# Autodesk Inventor assembly: V4Slapper
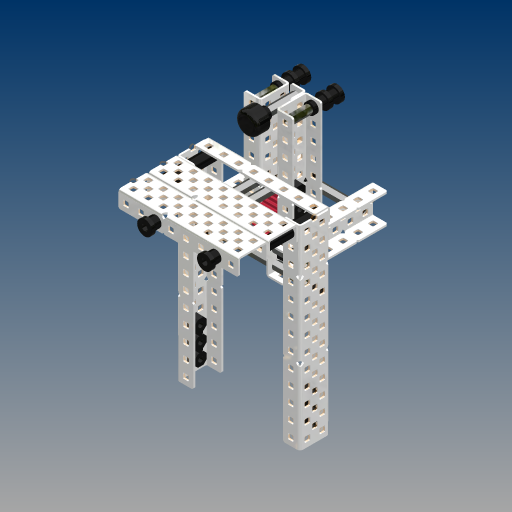
[picture p0: Inventor's stored thumbnail of the model, 512x512]
Saved by Autodesk Inventor 2023 (Build 270158000, 158)
## iProperties
Created: 2024-01-13
Part Number: V4Slapper
Document SubType Name: Assembly
Designer: eddie
Author: eddie
## Documents named in this file (24)
- C:\Users\eddie\Documents\81208X-Over-Under-CAD\V4\V4Slapper.iam
- C:\Users\eddie\Documents\81208X-Over-Under-CAD\VEX-CAD-Inventor-1.4.0\Structure\C Channel\Aluminum 1x2x1\Alu C 1x2x1x13.ipt
- C:\Users\eddie\Documents\81208X-Over-Under-CAD\VEX-CAD-Inventor-1.4.0\Motion\Spacers\Spacer Nylon .375 OD\NSpacer .375 OD x .500.ipt
- C:\Users\eddie\Documents\81208X-Over-Under-CAD\VEX-CAD-Inventor-1.4.0\Motion\Spacers\Spacer Nylon .375 OD.ipt
- C:\Users\eddie\Documents\81208X-Over-Under-CAD\VEX-CAD-Inventor-1.4.0\Structure\Standoff\Standoff 3.00.ipt
- C:\Users\eddie\Documents\81208X-Over-Under-CAD\VEX-CAD-Inventor-1.4.0\Structure\Standoff.ipt
- C:\Users\eddie\Documents\81208X-Over-Under-CAD\VEX-CAD-Inventor-1.4.0\Motion\Spacers\Spacer Nylon .375 OD\NSpacer .375 OD x .375.ipt
- C:\Users\eddie\Documents\81208X-Over-Under-CAD\VEX-CAD-Inventor-1.4.0\Structure\Angle\Aluminum\1x1\Alu Angle 1x1x8.ipt
- C:\Users\eddie\Documents\81208X-Over-Under-CAD\VEX-CAD-Inventor-1.4.0\Structure\C Channel\Aluminum 1x2x1\Alu C 1x2x1x8.ipt
- C:\Users\eddie\Documents\81208X-Over-Under-CAD\VEX-CAD-Inventor-1.4.0\Motion\Spacers\Spacer Nylon .375 OD\NSpacer .375 OD x .250.ipt
- C:\Users\eddie\Documents\81208X-Over-Under-CAD\VEX-CAD-Inventor-1.4.0\Motion\Spacers\Spacer Nylon .500 OD\NSpacer Black .500 OD x .125.ipt
- C:\Users\eddie\Documents\81208X-Over-Under-CAD\VEX-CAD-Inventor-1.4.0\Motion\Spacers\Spacer Nylon .500 OD.ipt
- C:\Users\eddie\Documents\81208X-Over-Under-CAD\VEX-CAD-Inventor-1.4.0\Motion\Shaft LS\Bearing Flat.ipt
- C:\Users\eddie\Documents\81208X-Over-Under-CAD\VEX-CAD-Inventor-1.4.0\Structure\Standoff\Standoff 1.00.ipt
- C:\Users\eddie\Documents\81208X-Over-Under-CAD\VEX-CAD-Inventor-1.4.0\Structure\C Channel\Aluminum 1x2x1\Alu C 1x2x1x7.ipt
- C:\Users\eddie\Documents\81208X-Over-Under-CAD\VEX-CAD-Inventor-1.4.0\Motion\Spacers\Washer Steel\SWasher .375 OD x .031250.ipt
- C:\Users\eddie\Documents\81208X-Over-Under-CAD\VEX-CAD-Inventor-1.4.0\Motion\Spacers\Washer Steel.ipt
- C:\Users\eddie\Documents\81208X-Over-Under-CAD\VEX-CAD-Inventor-1.4.0\Motion\Spacers\Spacer Nylon .375 OD\NSpacer .375 OD x .125.ipt
- C:\Users\eddie\Documents\81208X-Over-Under-CAD\VEX-CAD-Inventor-1.4.0\Structure\Standoff\Standoff 1.50.ipt
- C:\Users\eddie\Documents\81208X-Over-Under-CAD\VEX-CAD-Inventor-1.4.0\Motion\Gears\HS Gear\HS 36T Gear, Square.iam
- C:\Users\eddie\Documents\81208X-Over-Under-CAD\VEX-CAD-Inventor-1.4.0\Motion\Gears\HS Gear.iam
- C:\Users\eddie\Documents\81208X-Over-Under-CAD\VEX-CAD-Inventor-1.4.0\Structure\Standoff\Standoff .75.ipt
- C:\Users\eddie\Documents\81208X-Over-Under-CAD\VEX-CAD-Inventor-1.4.0\Structure\Angle\Aluminum\1x1\Alu Angle 1x1x3.ipt
- C:\Users\eddie\Documents\81208X-Over-Under-CAD\VEX-CAD-Inventor-1.4.0\Structure\Hardware\Rubber Bumper Threaded.ipt
## Components (61 placed, 18 different names)
1. Alu C 1x2x1x13:1 — Insert:2, Insert:5, Insert:9, Insert:10, Insert:22, Insert:25, Insert:26
2. Alu C 1x2x1x13:2 — Insert:1, Insert:6, Insert:20, Insert:21, Insert:23, Insert:24
3. NSpacer .375 OD x .500:1 — Insert:1, Insert:3
4. NSpacer .375 OD x .500:2 — Insert:2, Insert:4
5. Standoff 3.00:1 — Insert:3, Insert:4
6. NSpacer .375 OD x .500:3 — Insert:6, Insert:7
7. NSpacer .375 OD x .500:4 — Insert:5, Insert:8
8. NSpacer .375 OD x .375:5 — Insert:7
9. NSpacer .375 OD x .375:6 — Insert:8
10. Alu Angle 1x1x8:1 — Insert:9, Insert:27, Insert:28
11. Alu C 1x2x1x8:1 — Insert:10, Insert:11, Insert:12, Insert:14
12. Alu C 1x2x1x8:2 — Insert:11, Insert:16, Insert:17
13. NSpacer .375 OD x .500:7 — Insert:12, Insert:13
14. NSpacer .375 OD x .375:8 — Insert:13
15. NSpacer .375 OD x .500:9 — Insert:14, Insert:15
16. NSpacer .375 OD x .375:10 — Insert:15
17. NSpacer .375 OD x .250:11 — Insert:17, Insert:19
18. NSpacer .375 OD x .250:12 — Insert:16, Insert:18
19. NSpacer Black .500 OD x .125:1 — Insert:19
20. NSpacer Black .500 OD x .125:2 — Insert:18
21. Bearing Flat:1 — Insert:20, Insert:21
22. Bearing Flat:2 — Insert:22
23. Standoff 1.00:2 — Insert:24
24. Standoff 1.00:3 — Insert:23, Insert:30
25. Standoff 1.00:4 — Insert:25, Insert:29
26. Standoff 1.00:5 — Insert:26
27. Standoff 1.00:6 — Insert:28
28. Standoff 1.00:7 — Insert:27
29. Alu C 1x2x1x7:1 — Insert:30, Insert:33, Insert:35, Insert:44
30. Alu C 1x2x1x7:2 — Insert:29, Insert:32, Insert:34, Insert:43
31. Bearing Flat:4 — Insert:32
32. Bearing Flat:5 — Insert:33
33. SWasher .375 OD x .031250:1 — Insert:34, Insert:36
34. SWasher .375 OD x .031250:2 — Insert:35, Insert:37
35. NSpacer .375 OD x .125:13 — Insert:37, Insert:38
36. NSpacer .375 OD x .125:14 — Insert:36
37. Standoff 1.50:8 — Insert:38, Insert:39
38. NSpacer .375 OD x .125:15 — Insert:39
39. Alu C 1x2x1x8:3 — Insert:46, Insert:48, Insert:50, Insert:60, Insert:67
40. Alu C 1x2x1x8:4 — Insert:42, Insert:49, Insert:59
41. Bearing Flat:6 — Insert:42, Insert:45
42. NSpacer .375 OD x .375:18 — Insert:43, Insert:47
43. NSpacer .375 OD x .375:19 — Insert:44, Insert:45
44. Bearing Flat:7 — Insert:46, Insert:47
45. HS 36T Gear, Square:1 [sub-assembly] — Insert:48
46. Standoff .75:9 — Insert:50, Insert:52
47. Standoff .75:10 — Insert:49, Insert:51
48. NSpacer .375 OD x .125:20 — Insert:51
49. NSpacer .375 OD x .125:21 — Insert:52
50. NSpacer Black .500 OD x .125:5 — Insert:61, Insert:63
51. NSpacer Black .500 OD x .125:6 — Insert:62, Insert:64
52. NSpacer .375 OD x .250:26 — Insert:59, Insert:62
53. NSpacer .375 OD x .250:27 — Insert:60, Insert:61
54. NSpacer .375 OD x .250:28 — Insert:63, Insert:65
55. NSpacer .375 OD x .250:29 — Insert:64, Insert:66
56. NSpacer Black .500 OD x .125:7 — Insert:65
57. NSpacer Black .500 OD x .125:8 — Insert:66
58. Alu Angle 1x1x3:1 — Insert:67, Insert:68
59. Standoff 1.00:11 — Insert:68, Insert:69
60. NSpacer .375 OD x .250:30 — Insert:69, Insert:70
61. Rubber Bumper Threaded:1 — Insert:70
## Relationships (61: Insert 61)
- Insert:1: Alu C 1x2x1x13:2 ↔ NSpacer .375 OD x .500:1
- Insert:2: Alu C 1x2x1x13:1 ↔ NSpacer .375 OD x .500:2
- Insert:3: NSpacer .375 OD x .500:1 ↔ Standoff 3.00:1
- Insert:4: NSpacer .375 OD x .500:2 ↔ Standoff 3.00:1
- Insert:5: Alu C 1x2x1x13:1 ↔ NSpacer .375 OD x .500:4
- Insert:6: Alu C 1x2x1x13:2 ↔ NSpacer .375 OD x .500:3
- Insert:7: NSpacer .375 OD x .500:3 ↔ NSpacer .375 OD x .375:5
- Insert:8: NSpacer .375 OD x .500:4 ↔ NSpacer .375 OD x .375:6
- Insert:9: Alu C 1x2x1x13:1 ↔ Alu Angle 1x1x8:1
- Insert:10: Alu C 1x2x1x13:1 ↔ Alu C 1x2x1x8:1
- Insert:11: Alu C 1x2x1x8:1 ↔ Alu C 1x2x1x8:2
- Insert:12: Alu C 1x2x1x8:1 ↔ NSpacer .375 OD x .500:7
- Insert:13: NSpacer .375 OD x .500:7 ↔ NSpacer .375 OD x .375:8
- Insert:14: Alu C 1x2x1x8:1 ↔ NSpacer .375 OD x .500:9
- Insert:15: NSpacer .375 OD x .500:9 ↔ NSpacer .375 OD x .375:10
- Insert:16: Alu C 1x2x1x8:2 ↔ NSpacer .375 OD x .250:12
- Insert:17: Alu C 1x2x1x8:2 ↔ NSpacer .375 OD x .250:11
- Insert:18: NSpacer .375 OD x .250:12 ↔ NSpacer Black .500 OD x .125:2
- Insert:19: NSpacer .375 OD x .250:11 ↔ NSpacer Black .500 OD x .125:1
- Insert:20: Alu C 1x2x1x13:2 ↔ Bearing Flat:1
- Insert:21: Alu C 1x2x1x13:2 ↔ Bearing Flat:1
- Insert:22: Alu C 1x2x1x13:1 ↔ Bearing Flat:2
- Insert:23: Alu C 1x2x1x13:2 ↔ Standoff 1.00:3
- Insert:24: Alu C 1x2x1x13:2 ↔ Standoff 1.00:2
- Insert:25: Alu C 1x2x1x13:1 ↔ Standoff 1.00:4
- Insert:26: Alu C 1x2x1x13:1 ↔ Standoff 1.00:5
- Insert:27: Alu Angle 1x1x8:1 ↔ Standoff 1.00:7
- Insert:28: Alu Angle 1x1x8:1 ↔ Standoff 1.00:6
- Insert:29: Standoff 1.00:4 ↔ Alu C 1x2x1x7:2
- Insert:30: Standoff 1.00:3 ↔ Alu C 1x2x1x7:1
- Insert:32: Alu C 1x2x1x7:2 ↔ Bearing Flat:4
- Insert:33: Alu C 1x2x1x7:1 ↔ Bearing Flat:5
- Insert:34: Alu C 1x2x1x7:2 ↔ SWasher .375 OD x .031250:1
- Insert:35: Alu C 1x2x1x7:1 ↔ SWasher .375 OD x .031250:2
- Insert:36: SWasher .375 OD x .031250:1 ↔ NSpacer .375 OD x .125:14
- Insert:37: SWasher .375 OD x .031250:2 ↔ NSpacer .375 OD x .125:13
- Insert:38: NSpacer .375 OD x .125:13 ↔ Standoff 1.50:8
- Insert:39: Standoff 1.50:8 ↔ NSpacer .375 OD x .125:15
- Insert:42: Alu C 1x2x1x8:4 ↔ Bearing Flat:6
- Insert:43: Alu C 1x2x1x7:2 ↔ NSpacer .375 OD x .375:18
- Insert:44: Alu C 1x2x1x7:1 ↔ NSpacer .375 OD x .375:19
- Insert:45: Bearing Flat:6 ↔ NSpacer .375 OD x .375:19
- Insert:46: Alu C 1x2x1x8:3 ↔ Bearing Flat:7
- Insert:47: NSpacer .375 OD x .375:18 ↔ Bearing Flat:7
- Insert:48: Alu C 1x2x1x8:3 ↔ HS 36T Gear, Square:1
- Insert:49: Alu C 1x2x1x8:4 ↔ Standoff .75:10
- Insert:50: Alu C 1x2x1x8:3 ↔ Standoff .75:9
- Insert:51: Standoff .75:10 ↔ NSpacer .375 OD x .125:20
- Insert:52: Standoff .75:9 ↔ NSpacer .375 OD x .125:21
- Insert:59: Alu C 1x2x1x8:4 ↔ NSpacer .375 OD x .250:26
- Insert:60: Alu C 1x2x1x8:3 ↔ NSpacer .375 OD x .250:27
- Insert:61: NSpacer Black .500 OD x .125:5 ↔ NSpacer .375 OD x .250:27
- Insert:62: NSpacer Black .500 OD x .125:6 ↔ NSpacer .375 OD x .250:26
- Insert:63: NSpacer Black .500 OD x .125:5 ↔ NSpacer .375 OD x .250:28
- Insert:64: NSpacer Black .500 OD x .125:6 ↔ NSpacer .375 OD x .250:29
- Insert:65: NSpacer .375 OD x .250:28 ↔ NSpacer Black .500 OD x .125:7
- Insert:66: NSpacer .375 OD x .250:29 ↔ NSpacer Black .500 OD x .125:8
- Insert:67: Alu C 1x2x1x8:3 ↔ Alu Angle 1x1x3:1
- Insert:68: Alu Angle 1x1x3:1 ↔ Standoff 1.00:11
- Insert:69: Standoff 1.00:11 ↔ NSpacer .375 OD x .250:30
- Insert:70: NSpacer .375 OD x .250:30 ↔ Rubber Bumper Threaded:1
